# Autodesk Inventor assembly: ElevDriveShaft
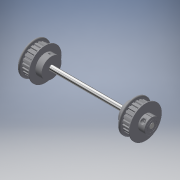
[picture p0: Inventor's stored thumbnail of the model, 180x180]
Saved by Autodesk Inventor 2019 (Build 230136000, 136)
## iProperties
Created: 2019-09-28
Part Number: ElevDriveShaft
Document SubType Name: Assembly
Designer: james
Author: james
## Documents named in this file (4)
- F:\JimsDesign\Jims2020FTC\ElevDriveShaft.iam
- F:\JimsDesign\Jims2020FTC\ElevatorShaft.ipt
- F:\JimsDesign\Library\McMaster\57445K230_ONE-PIECE CLAMP-ON SHAFT COLLAR.ipt
- F:\JimsDesign\Library\McMaster\TimingBelt\6495K721_TIMING BELT PULLEY.ipt
## Components (5 placed, 3 different names)
1. ElevatorShaft:1 — Mate:1, Mate:2, Flush:1, Flush:2
2. 57445K230_ONE-PIECE CLAMP-ON SHAFT COLLAR:1 — Mate:1, Flush:2
3. 57445K230_ONE-PIECE CLAMP-ON SHAFT COLLAR:2 — Mate:2, Flush:1
4. 6495K721_TIMING BELT PULLEY:1
5. 6495K721_TIMING BELT PULLEY:2
## Relationships (6: Mate 4, Flush 2)
- Mate:1: ElevatorShaft:1 ↔ 57445K230_ONE-PIECE CLAMP-ON SHAFT COLLAR:1
- Mate:2: ElevatorShaft:1 ↔ 57445K230_ONE-PIECE CLAMP-ON SHAFT COLLAR:2
- Flush:1: ElevatorShaft:1 ↔ 57445K230_ONE-PIECE CLAMP-ON SHAFT COLLAR:2
- Flush:2: ElevatorShaft:1 ↔ 57445K230_ONE-PIECE CLAMP-ON SHAFT COLLAR:1
- [Mate]: ElevatorShaft:1 ↔ 6495K721_TIMING BELT PULLEY:2
- [Mate]: ElevatorShaft:1 ↔ 6495K721_TIMING BELT PULLEY:1
